# Autodesk Inventor assembly: ASM Printing Head
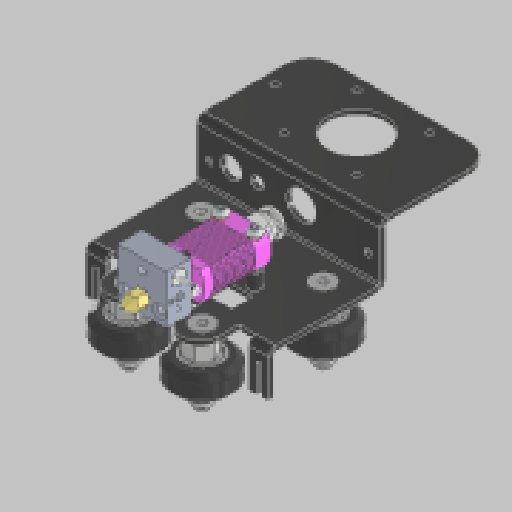
[picture p0: Inventor's stored thumbnail of the model, 512x512]
Saved by Autodesk Inventor 2025.3 (Build 293356000, 356)
## iProperties
Created: 2022-04-13
Part Number: ASM Printing Head
Document SubType Name: Assembly
Designer: javie
Author: javie
Revision Number: ANY
## Documents named in this file (8)
- C:\Users\Inema\OneDrive - INEMA S.A\Escritorio\Modelo Ender 3\ASM Printing Head.iam
- C:\Users\Inema\OneDrive - INEMA S.A\Escritorio\Modelo Ender 3\E plate.ipt
- C:\Users\Inema\OneDrive - INEMA S.A\Escritorio\Modelo Ender 3\Fan cover.ipt
- C:\Users\Inema\OneDrive - INEMA S.A\Escritorio\Modelo Ender 3\Nozzle fan duct.ipt
- C:\Users\Inema\OneDrive - INEMA S.A\Escritorio\Modelo Ender 3\ASM Heating Unit.iam
- C:\Users\Inema\OneDrive - INEMA S.A\Escritorio\Modelo Ender 3\ASM Roller X-Axis.iam
- C:\Users\Inema\OneDrive - INEMA S.A\Escritorio\Modelo Ender 3\ASM Eccentrical Roller X-Axis.iam
- C:\Users\Inema\OneDrive - INEMA S.A\Escritorio\Modelo Ender 3\CARRO ENDER3 -CR10\CARRO ENDER3 -CR10\CARRO ENDER3 -CR10.iam
## Components (8 placed, 8 different names)
1. E plate_168 — Coincidencia:1, Coincidencia:2, Nivelación:1, Coincidencia:3
2. Fan cover_170 — Coincidencia:1, Coincidencia:2, Nivelación:1, Nivelación:2, Coincidencia:4
3. Nozzle fan duct_171
4. ASM Heating Unit_173 [sub-assembly] — Coincidencia:3, Nivelación:2, Coincidencia:4, Ángulo:1, Insertar:1, Coincidencia:8
5. ASM Roller X-Axis_174 [sub-assembly]
6. ASM Roller X-Axis_175 [sub-assembly]
7. ASM Eccentrical Roller X-Axis_176 [sub-assembly]
8. CARRO ENDER3 -CR10:1 [sub-assembly] — Ángulo:1, Insertar:1, Coincidencia:8
## Relationships (9: Mate 5, Flush 2, Angle 1, Insert 1)
- Coincidencia:1 [Mate]: E plate_168 ↔ Fan cover_170
- Coincidencia:2 [Mate]: E plate_168 ↔ Fan cover_170
- Nivelación:1 [Flush] (-45.3 mm): E plate_168 ↔ Fan cover_170
- Coincidencia:3 [Mate] (0.8 mm): E plate_168 ↔ ASM Heating Unit_173
- Nivelación:2 [Flush] (-18 mm): Fan cover_170 ↔ ASM Heating Unit_173
- Coincidencia:4 [Mate] (-49.35 mm): Fan cover_170 ↔ ASM Heating Unit_173
- Ángulo:1 [Angle] (180 deg): ASM Heating Unit_173 ↔ CARRO ENDER3 -CR10:1
- Insertar:1: ASM Heating Unit_173 ↔ CARRO ENDER3 -CR10:1
- Coincidencia:8 [Mate]: ASM Heating Unit_173 ↔ CARRO ENDER3 -CR10:1
